# Autodesk Inventor assembly: 6P Sprocket
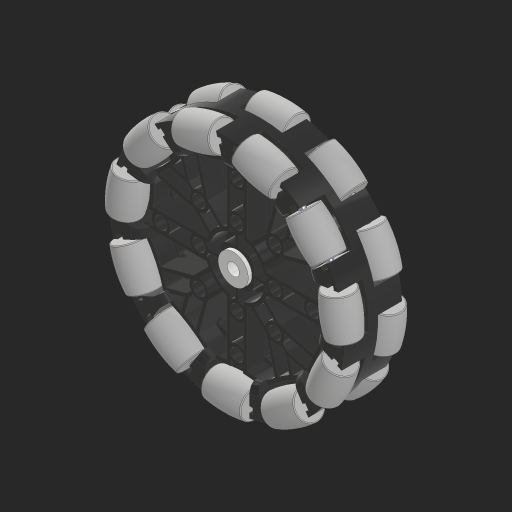
[picture p0: Inventor's stored thumbnail of the model, 512x512]
Saved by Autodesk Inventor 2023 (Build 270158000, 158)
## iProperties
Created: 2022-08-02
Part Number: 6P Sprocket
Document SubType Name: Assembly
Designer: ylu12
Author: ylu12
## Documents named in this file (4)
- C:\Users\ylu12\Documents\GitHub\VEX-CAD-Inventor\Motion\Wheels\Omni Wheel\3.25 Omni AS, Circle.iam
- C:\Users\ylu12\Documents\GitHub\VEX-CAD-Inventor\Motion\Wheels\Reference Files\3.25 Omni Antistatic.ipt
- C:\Users\ylu12\Documents\GitHub\VEX-CAD-Inventor\Motion\Insert Circle.ipt
- C:\Users\ylu12\Documents\GitHub\VEX-CAD-Inventor\Motion\Wheels\Omni Wheel.iam
## Components (3 placed, 3 different names)
1. 3.25 Omni Antistatic
2. Circle 1 — Flush:12, Flush:13, Flush:14, Mate:20, Angle:2
3. Circle 2 — Flush:12, Flush:13, Mate:19
## Relationships (9: Flush 4, Mate 4, Angle 1)
- [Flush]: 3.25 Omni Antistatic
- [Mate]: 3.25 Omni Antistatic
- [Mate]: 3.25 Omni Antistatic
- Flush:12: Circle 1 ↔ Circle 2
- Flush:13: Circle 1 ↔ Circle 2
- Mate:19 (6.35 mm): Circle 2
- Flush:14 (6.35 mm): Circle 1
- Mate:20: Circle 1
- Angle:2 (0 deg): Circle 1
## Named parameters: HalfWheelWidth = 6.35 mm
